# Autodesk Inventor assembly: Kinematic-Mount Front [B]
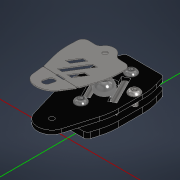
[picture p0: Inventor's stored thumbnail of the model, 180x180]
Saved by Autodesk Inventor 2022.2 (Build 262287010, 287A)
## iProperties
Created: 2022-03-13
Part Number: Kinematic-Mount Front [B]
Document SubType Name: Assembly
Designer: sleib
Author: sleib
## Documents named in this file (9)
- C:\Users\sleib\Projekte\Voron-2\CAD\Inventor\Kinematic-Mount Front [B].iam
- C:\Users\sleib\Projekte\Voron-2\CAD\Inventor\Kinematic-Bed Front-Support Bottom.ipt
- C:\Users\sleib\Projekte\Voron-2\CAD\Inventor\Pin 5x15.ipt
- C:\Users\sleib\Projekte\Voron-2\CAD\Inventor\Kinematic-Bed Front-Support Top.ipt
- C:\Users\sleib\Projekte\Voron-2\CAD\Inventor\M3x8 BHCS.ipt
- C:\Users\sleib\Projekte\Voron-2\CAD\Inventor\M3x12 BHCS.ipt
- C:\Users\sleib\Projekte\Voron-2\CAD\Inventor\M3 Threaded Ball.ipt
- C:\Users\sleib\Projekte\Voron-2\CAD\Inventor\M3x10x6 Standoff.ipt
- C:\Users\sleib\Projekte\Voron-2\CAD\Inventor\Kinematic-Bed Leaf-Spring.ipt
## Components (11 placed, 8 different names)
1. Kinematic-Bed Front-Support Bottom:1 — Passend:1, Passend:2, Passend:3, Passend:4, Passend:30, Passend:31, Passend:32, Passend:33, Passend:34, Passend:35, Passend:37, Passend:39, Passend:41, Passend:43
2. Kinematic-Bed Front-Support Top:1 — Passend:11, Passend:12, Passend:29, Passend:36, Passend:38, Passend:40, Passend:42, Passend:44, Passend:45, Passend:46, Passend:47
3. Kinematic-Bed Leaf-Spring:1 — Passend:27, Passend:28, Passend:29
4. M3 Threaded Ball:1 — Tangential:1, Tangential:2, Passend:25, Passend:26
5. M3x10x6 Standoff:1 — Passend:25, Passend:26, Passend:27, Passend:28
6. Pin 5x15:1 — Passend:30, Passend:31, Passend:34, Passend:11, Tangential:2
7. Pin 5x15:2 — Passend:32, Passend:33, Passend:35, Passend:12, Tangential:1
8. M3x8 BHCS:3 — Passend:40, Passend:41, Passend:46
9. M3x8 BHCS:4 — Passend:42, Passend:43, Passend:44
10. M3x12 BHCS:1 — Passend:38, Passend:39, Passend:45
11. M3x12 BHCS:2 — Passend:36, Passend:37, Passend:47
## Relationships (31: Mate 29, Tangent 2)
- Passend:1 [Mate]: Kinematic-Bed Front-Support Bottom:1
- Passend:2 [Mate]: Kinematic-Bed Front-Support Bottom:1
- Passend:3 [Mate]: Kinematic-Bed Front-Support Bottom:1
- Passend:4 [Mate]: Kinematic-Bed Front-Support Bottom:1
- Passend:30 [Mate] (2.5 mm): Kinematic-Bed Front-Support Bottom:1 ↔ Pin 5x15:1
- Passend:31 [Mate] (2.5 mm): Kinematic-Bed Front-Support Bottom:1 ↔ Pin 5x15:1
- Passend:34 [Mate] (0.2 mm): Kinematic-Bed Front-Support Bottom:1 ↔ Pin 5x15:1
- Passend:11 [Mate] (2.5 mm): Kinematic-Bed Front-Support Top:1 ↔ Pin 5x15:1
- Passend:32 [Mate] (2.5 mm): Kinematic-Bed Front-Support Bottom:1 ↔ Pin 5x15:2
- Passend:33 [Mate] (2.5 mm): Kinematic-Bed Front-Support Bottom:1 ↔ Pin 5x15:2
- Passend:35 [Mate] (0.2 mm): Kinematic-Bed Front-Support Bottom:1 ↔ Pin 5x15:2
- Passend:12 [Mate] (2.5 mm): Kinematic-Bed Front-Support Top:1 ↔ Pin 5x15:2
- Tangential:1: M3 Threaded Ball:1 ↔ Pin 5x15:2
- Tangential:2: M3 Threaded Ball:1 ↔ Pin 5x15:1
- Passend:25 [Mate]: M3 Threaded Ball:1 ↔ M3x10x6 Standoff:1
- Passend:26 [Mate] (1 mm): M3 Threaded Ball:1 ↔ M3x10x6 Standoff:1
- Passend:27 [Mate]: Kinematic-Bed Leaf-Spring:1 ↔ M3x10x6 Standoff:1
- Passend:28 [Mate]: Kinematic-Bed Leaf-Spring:1 ↔ M3x10x6 Standoff:1
- Passend:29 [Mate]: Kinematic-Bed Front-Support Top:1 ↔ Kinematic-Bed Leaf-Spring:1
- Passend:36 [Mate]: Kinematic-Bed Front-Support Top:1 ↔ M3x12 BHCS:2
- Passend:37 [Mate]: Kinematic-Bed Front-Support Bottom:1 ↔ M3x12 BHCS:2
- Passend:38 [Mate]: Kinematic-Bed Front-Support Top:1 ↔ M3x12 BHCS:1
- Passend:39 [Mate]: Kinematic-Bed Front-Support Bottom:1 ↔ M3x12 BHCS:1
- Passend:40 [Mate]: Kinematic-Bed Front-Support Top:1 ↔ M3x8 BHCS:3
- Passend:41 [Mate]: Kinematic-Bed Front-Support Bottom:1 ↔ M3x8 BHCS:3
- Passend:42 [Mate]: Kinematic-Bed Front-Support Top:1 ↔ M3x8 BHCS:4
- Passend:43 [Mate]: Kinematic-Bed Front-Support Bottom:1 ↔ M3x8 BHCS:4
- Passend:44 [Mate]: Kinematic-Bed Front-Support Top:1 ↔ M3x8 BHCS:4
- Passend:45 [Mate]: Kinematic-Bed Front-Support Top:1 ↔ M3x12 BHCS:1
- Passend:46 [Mate]: Kinematic-Bed Front-Support Top:1 ↔ M3x8 BHCS:3
- Passend:47 [Mate]: Kinematic-Bed Front-Support Top:1 ↔ M3x12 BHCS:2
